# Autodesk Inventor assembly: AMR_Base
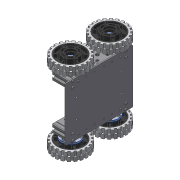
[picture p0: Inventor's stored thumbnail of the model, 180x180]
Saved by Autodesk Inventor 2018 (Build 220112000, 112)
## iProperties
Created: 2019-08-30
Part Number: AMR_Base
Document SubType Name: Assembly
Designer: Clevo
Author: Clevo
## Documents named in this file (8)
- E:\Hardware_Accelerated_Robot\Hardware\AMR_Base.iam
- E:\Hardware_Accelerated_Robot\Hardware\AMR_Transm.iam
- E:\Hardware_Accelerated_Robot\Hardware\AMR_Transm2.iam
- E:\Hardware_Accelerated_Robot\Hardware\CustomParts\Battery_Base.ipt
- E:\Hardware_Accelerated_Robot\Hardware\Extrusions\1050-2-CL.ipt
- E:\Hardware_Accelerated_Robot\Hardware\Wheels\94500A232_TYPE 316 SS BUTTON-HEAD SOCKET CAP SCREW.ipt
- E:\Hardware_Accelerated_Robot\Hardware\Wheels\94500A226_TYPE 316 SS BUTTON-HEAD SOCKET CAP SCREW.ipt
- E:\Hardware_Accelerated_Robot\Hardware\CustomParts\Battery_Base_ForPrint.ipt
## Components (22 placed, 7 different names)
1. AMR_Transm:1 [sub-assembly] — Flush:1, Flush:2, Flush:7, Mate:2
2. AMR_Transm2:1 [sub-assembly] — Flush:1, Flush:2, Flush:5, Flush:6, Mate:1
3. AMR_Transm:2 [sub-assembly] — Flush:5, Flush:6, Mate:3, Mate:4
4. AMR_Transm2:2 [sub-assembly] — Flush:7
5. Battery_Base:1 — Mate:1, Mate:2, Mate:3, Mate:4, Mate:5, Mate:6, Mate:7, Mate:8, Mate:9, Mate:10, Mate:11, Mate:12, Mate:13, Mate:14, Mate:15, Mate:16, Mate:17, Mate:18, Mate:19, Mate:20, Mate:21, Mate:22, Mate:23, Mate:24, Mate:25, Mate:26, Mate:27, Mate:28, Mate:29, Mate:30, Mate:31, Mate:32, Mate:33, Mate:34, Mate:35, Mate:36, Mate:37, Mate:38, Mate:39, Mate:40, Flush:8, Flush:9, Flush:10
6. 1050-2-CL:1 — Mate:5, Mate:6, Mate:7
7. 1050-2-CL:2 — Mate:11, Mate:12, Mate:13
8. 1050-2-CL:3 — Mate:8, Mate:9, Mate:10
9. 1050-2-CL:4 — Mate:14, Mate:15, Mate:16
10. 94500A232_TYPE 316 SS BUTTON-HEAD SOCKET CAP SCREW:1 — Mate:17, Mate:26
11. 94500A226_TYPE 316 SS BUTTON-HEAD SOCKET CAP SCREW:1 — Mate:36, Mate:39
12. 94500A232_TYPE 316 SS BUTTON-HEAD SOCKET CAP SCREW:2 — Mate:18, Mate:25
13. 94500A232_TYPE 316 SS BUTTON-HEAD SOCKET CAP SCREW:3 — Mate:20, Mate:28
14. 94500A232_TYPE 316 SS BUTTON-HEAD SOCKET CAP SCREW:4 — Mate:19, Mate:27
15. 94500A232_TYPE 316 SS BUTTON-HEAD SOCKET CAP SCREW:5 — Mate:22, Mate:29
16. 94500A232_TYPE 316 SS BUTTON-HEAD SOCKET CAP SCREW:6 — Mate:21, Mate:30
17. 94500A232_TYPE 316 SS BUTTON-HEAD SOCKET CAP SCREW:7 — Mate:24, Mate:32
18. 94500A232_TYPE 316 SS BUTTON-HEAD SOCKET CAP SCREW:8 — Mate:23, Mate:31
19. 94500A226_TYPE 316 SS BUTTON-HEAD SOCKET CAP SCREW:2 — Mate:35, Mate:40
20. 94500A226_TYPE 316 SS BUTTON-HEAD SOCKET CAP SCREW:3 — Mate:34, Mate:38
21. 94500A226_TYPE 316 SS BUTTON-HEAD SOCKET CAP SCREW:4 — Mate:33, Mate:37
22. Battery_Base_ForPrint:1 — Flush:8, Flush:9, Flush:10
## Relationships (50: Mate 40, Flush 10)
- Flush:1: AMR_Transm:1 ↔ AMR_Transm2:1
- Flush:2: AMR_Transm:1 ↔ AMR_Transm2:1
- [Flush]: AMR_Transm:2 ↔ AMR_Transm2:2
- [Flush]: AMR_Transm:2 ↔ AMR_Transm2:2
- Flush:5: AMR_Transm2:1 ↔ AMR_Transm:2
- Flush:6: AMR_Transm2:1 ↔ AMR_Transm:2
- Flush:7: AMR_Transm:1 ↔ AMR_Transm2:2
- Mate:1: AMR_Transm2:1 ↔ Battery_Base:1
- Mate:2: AMR_Transm:1 ↔ Battery_Base:1
- Mate:3: AMR_Transm:2 ↔ Battery_Base:1
- Mate:4: AMR_Transm:2 ↔ Battery_Base:1
- Mate:5: Battery_Base:1 ↔ 1050-2-CL:1
- Mate:6: Battery_Base:1 ↔ 1050-2-CL:1
- Mate:7: Battery_Base:1 ↔ 1050-2-CL:1
- Mate:8: Battery_Base:1 ↔ 1050-2-CL:3
- Mate:9: Battery_Base:1 ↔ 1050-2-CL:3
- Mate:10: Battery_Base:1 ↔ 1050-2-CL:3
- Mate:11: Battery_Base:1 ↔ 1050-2-CL:2
- Mate:12: Battery_Base:1 ↔ 1050-2-CL:2
- Mate:13: Battery_Base:1 ↔ 1050-2-CL:2
- Mate:14: Battery_Base:1 ↔ 1050-2-CL:4
- Mate:15: Battery_Base:1 ↔ 1050-2-CL:4
- Mate:16: Battery_Base:1 ↔ 1050-2-CL:4
- Mate:17: Battery_Base:1 ↔ 94500A232_TYPE 316 SS BUTTON-HEAD SOCKET CAP SCREW:1
- Mate:18: Battery_Base:1 ↔ 94500A232_TYPE 316 SS BUTTON-HEAD SOCKET CAP SCREW:2
- Mate:19: Battery_Base:1 ↔ 94500A232_TYPE 316 SS BUTTON-HEAD SOCKET CAP SCREW:4
- Mate:20: Battery_Base:1 ↔ 94500A232_TYPE 316 SS BUTTON-HEAD SOCKET CAP SCREW:3
- Mate:21: Battery_Base:1 ↔ 94500A232_TYPE 316 SS BUTTON-HEAD SOCKET CAP SCREW:6
- Mate:22: Battery_Base:1 ↔ 94500A232_TYPE 316 SS BUTTON-HEAD SOCKET CAP SCREW:5
- Mate:23: Battery_Base:1 ↔ 94500A232_TYPE 316 SS BUTTON-HEAD SOCKET CAP SCREW:8
- Mate:24: Battery_Base:1 ↔ 94500A232_TYPE 316 SS BUTTON-HEAD SOCKET CAP SCREW:7
- Mate:25: Battery_Base:1 ↔ 94500A232_TYPE 316 SS BUTTON-HEAD SOCKET CAP SCREW:2
- Mate:26: Battery_Base:1 ↔ 94500A232_TYPE 316 SS BUTTON-HEAD SOCKET CAP SCREW:1
- Mate:27: Battery_Base:1 ↔ 94500A232_TYPE 316 SS BUTTON-HEAD SOCKET CAP SCREW:4
- Mate:28: Battery_Base:1 ↔ 94500A232_TYPE 316 SS BUTTON-HEAD SOCKET CAP SCREW:3
- Mate:29: Battery_Base:1 ↔ 94500A232_TYPE 316 SS BUTTON-HEAD SOCKET CAP SCREW:5
- Mate:30: Battery_Base:1 ↔ 94500A232_TYPE 316 SS BUTTON-HEAD SOCKET CAP SCREW:6
- Mate:31: Battery_Base:1 ↔ 94500A232_TYPE 316 SS BUTTON-HEAD SOCKET CAP SCREW:8
- Mate:32: Battery_Base:1 ↔ 94500A232_TYPE 316 SS BUTTON-HEAD SOCKET CAP SCREW:7
- Mate:33: Battery_Base:1 ↔ 94500A226_TYPE 316 SS BUTTON-HEAD SOCKET CAP SCREW:4
- Mate:34: Battery_Base:1 ↔ 94500A226_TYPE 316 SS BUTTON-HEAD SOCKET CAP SCREW:3
- Mate:35: Battery_Base:1 ↔ 94500A226_TYPE 316 SS BUTTON-HEAD SOCKET CAP SCREW:2
- Mate:36: Battery_Base:1 ↔ 94500A226_TYPE 316 SS BUTTON-HEAD SOCKET CAP SCREW:1
- Mate:37: Battery_Base:1 ↔ 94500A226_TYPE 316 SS BUTTON-HEAD SOCKET CAP SCREW:4
- Mate:38: Battery_Base:1 ↔ 94500A226_TYPE 316 SS BUTTON-HEAD SOCKET CAP SCREW:3
- Mate:39: Battery_Base:1 ↔ 94500A226_TYPE 316 SS BUTTON-HEAD SOCKET CAP SCREW:1
- Mate:40: Battery_Base:1 ↔ 94500A226_TYPE 316 SS BUTTON-HEAD SOCKET CAP SCREW:2
- Flush:8: Battery_Base:1 ↔ Battery_Base_ForPrint:1
- Flush:9: Battery_Base:1 ↔ Battery_Base_ForPrint:1
- Flush:10: Battery_Base:1 ↔ Battery_Base_ForPrint:1
## Named parameters: d14_d12 = 0 mm, d15_d13 = 0 mm
